# Autodesk Inventor assembly: Pendolo_Inverso
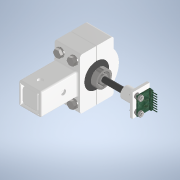
[picture p0: Inventor's stored thumbnail of the model, 180x180]
Saved by Autodesk Inventor 2020.2 (Build 242310000, 310)
## iProperties
Created: 2019-11-10
Part Number: Pendolo_Inverso
Document SubType Name: Assembly
Designer: socci
Author: socci
## Documents named in this file (12)
- C:\Users\socci\Desktop\mv-Project\04_PartDraw\Assieme_Connettore_Inferiore.iam
- C:\Users\socci\Documents\Inventor\Content Center Files\R2020\it-IT\Bearing GB_T 5800-2003\Rolling bearing GB_T 5800-2003 -635.ipt
- C:\Users\socci\Desktop\mv-Project\04_PartDraw\Componenti\1_Asse_cuscinetti.ipt
- C:\Users\socci\Desktop\mv-Project\04_PartDraw\Componenti\2_Connettore_inf_sup.ipt
- C:\Users\socci\Desktop\mv-Project\04_PartDraw\Componenti\3_Connettore_inf_INF.ipt
- C:\Users\socci\Desktop\mv-Project\04_PartDraw\Componenti\11_Connettore_MPU.ipt
- C:\Users\socci\Desktop\mv-Project\04_PartDraw\Componenti\10_MPU_6050.ipt
- C:\Users\socci\Documents\Inventor\Content Center Files\R2020\it-IT\UNI 5739\UNI 5739 - M5 x 40.ipt
- C:\Users\socci\Documents\Inventor\Content Center Files\R2020\it-IT\IS 2016  A\IS 2016 - A5,5.ipt
- C:\Users\socci\Documents\Inventor\Content Center Files\R2020\it-IT\AS 1112 (4)\AS 1112 - M5(2).ipt
- C:\Users\socci\Documents\Inventor\Content Center Files\R2020\it-IT\AS 1112 (2)\AS 1112 - M3  Tipo 5.ipt
- C:\Users\socci\Documents\Inventor\Content Center Files\R2020\it-IT\AS 1110\AS 1110 - M3 x 10.ipt
## Components (29 placed, 11 different names)
1. Bearing GB/T 5800-2003 635:1 — Inserimento:3
2. Bearing GB/T 5800-2003 635:2 — Inserimento:4
3. 1_Asse_cuscinetti:1 — Inserimento:3, Inserimento:4, Inserimento:5, Inserimento:6, Inserimento:7
4. 2_Connettore_inf_sup:1 — Inserimento:6, Coincidente:1, Allineato:3, Inserimento:337, Inserimento:338, Inserimento:341, Inserimento:342, Inserimento:345, Inserimento:346, Inserimento:349, Inserimento:350, Coincidente:3, Coincidente:4
5. 3_Connettore_inf_INF:1 — Inserimento:5, Coincidente:1, Inserimento:343, Inserimento:347, Inserimento:351, Inserimento:339
6. 11_Connettore_MPU:1 — Coincidente:2, Allineato:1, Allineato:2, Allineato:3, Inserimento:7
7. 10_MPU_6050:1 — Coincidente:2, Allineato:1, Allineato:2, Inserimento:373, Inserimento:374, Inserimento:375, Inserimento:376
8. AS 1112 (2) - Metrico M3  Tipo 5:6 — Inserimento:374, Inserimento:377
9. AS 1110 - Metrico M3 x 10:1 — Inserimento:377
10. AS 1112 (2) - Metrico M3  Tipo 5:5 — Inserimento:373
11. AS 1110 - Metrico M3 x 10:2 — Inserimento:378
12. AS 1112 (2) - Metrico M3  Tipo 5:7 — Inserimento:375
13. AS 1112 (2) - Metrico M3  Tipo 5:8 — Inserimento:376, Inserimento:378
14. UNI 5739 M5 x 40:8
15. IS 2016 A A5,5:15 — Inserimento:338
16. IS 2016 A A5,5:16 — Inserimento:337
17. AS 1112 (4) - Metrico M5:5 — Inserimento:339
18. UNI 5739 M5 x 40:9
19. IS 2016 A A5,5:17 — Inserimento:342
20. IS 2016 A A5,5:18 — Inserimento:341
21. AS 1112 (4) - Metrico M5:6 — Inserimento:343
22. UNI 5739 M5 x 40:10
23. IS 2016 A A5,5:19 — Inserimento:346
24. IS 2016 A A5,5:20 — Inserimento:345
25. AS 1112 (4) - Metrico M5:7 — Inserimento:347
26. UNI 5739 M5 x 40:11
27. IS 2016 A A5,5:21 — Inserimento:350
28. IS 2016 A A5,5:22 — Inserimento:349
29. AS 1112 (4) - Metrico M5:8 — Inserimento:351
## Relationships (34: Insert 27, Mate 4, Flush 3)
- Inserimento:3 (1.5 mm): Bearing GB/T 5800-2003 635:1 ↔ 1_Asse_cuscinetti:1
- Inserimento:4 (2.5 mm): Bearing GB/T 5800-2003 635:2 ↔ 1_Asse_cuscinetti:1
- Inserimento:5: 1_Asse_cuscinetti:1 ↔ 3_Connettore_inf_INF:1
- Inserimento:6: 1_Asse_cuscinetti:1 ↔ 2_Connettore_inf_sup:1
- Coincidente:1 [Mate] (1 mm): 2_Connettore_inf_sup:1 ↔ 3_Connettore_inf_INF:1
- Coincidente:2 [Mate] (2.4 mm): 11_Connettore_MPU:1 ↔ 10_MPU_6050:1
- Allineato:1 [Flush] (2 mm): 11_Connettore_MPU:1 ↔ 10_MPU_6050:1
- Allineato:2 [Flush] (3 mm): 11_Connettore_MPU:1 ↔ 10_MPU_6050:1
- Allineato:3 [Flush] (-9.5 mm): 2_Connettore_inf_sup:1 ↔ 11_Connettore_MPU:1
- Inserimento:7: 1_Asse_cuscinetti:1 ↔ 11_Connettore_MPU:1
- [Insert]: UNI 5739 M5 x 40:8 ↔ IS 2016 A A5,5:16
- Inserimento:337: 2_Connettore_inf_sup:1 ↔ IS 2016 A A5,5:16
- Inserimento:338: 2_Connettore_inf_sup:1 ↔ IS 2016 A A5,5:15
- Inserimento:339: 3_Connettore_inf_INF:1 ↔ AS 1112 (4) - Metrico M5:5
- [Insert]: UNI 5739 M5 x 40:9 ↔ IS 2016 A A5,5:18
- Inserimento:341: 2_Connettore_inf_sup:1 ↔ IS 2016 A A5,5:18
- Inserimento:342: 2_Connettore_inf_sup:1 ↔ IS 2016 A A5,5:17
- Inserimento:343: 3_Connettore_inf_INF:1 ↔ AS 1112 (4) - Metrico M5:6
- [Insert]: UNI 5739 M5 x 40:10 ↔ IS 2016 A A5,5:20
- Inserimento:345: 2_Connettore_inf_sup:1 ↔ IS 2016 A A5,5:20
- Inserimento:346: 2_Connettore_inf_sup:1 ↔ IS 2016 A A5,5:19
- Inserimento:347: 3_Connettore_inf_INF:1 ↔ AS 1112 (4) - Metrico M5:7
- [Insert]: UNI 5739 M5 x 40:11 ↔ IS 2016 A A5,5:22
- Inserimento:349: 2_Connettore_inf_sup:1 ↔ IS 2016 A A5,5:22
- Inserimento:350: 2_Connettore_inf_sup:1 ↔ IS 2016 A A5,5:21
- Inserimento:351: 3_Connettore_inf_INF:1 ↔ AS 1112 (4) - Metrico M5:8
- Inserimento:373: 10_MPU_6050:1 ↔ AS 1112 (2) - Metrico M3  Tipo 5:5
- Inserimento:374: 10_MPU_6050:1 ↔ AS 1112 (2) - Metrico M3  Tipo 5:6
- Inserimento:375: 10_MPU_6050:1 ↔ AS 1112 (2) - Metrico M3  Tipo 5:7
- Inserimento:376: 10_MPU_6050:1 ↔ AS 1112 (2) - Metrico M3  Tipo 5:8
- Inserimento:377 (3 mm): AS 1112 (2) - Metrico M3  Tipo 5:6 ↔ AS 1110 - Metrico M3 x 10:1
- Inserimento:378 (3 mm): AS 1110 - Metrico M3 x 10:2 ↔ AS 1112 (2) - Metrico M3  Tipo 5:8
- Coincidente:3 [Mate]: 2_Connettore_inf_sup:1
- Coincidente:4 [Mate]: 2_Connettore_inf_sup:1
## Named parameters: d535_d530_d518 = 0 mm, d539_d530_d518 = 0 mm, d543_d530_d518 = 0 mm, d547_d530_d518 = 0 mm
